# Autodesk Inventor assembly: Lower_Leg_Right
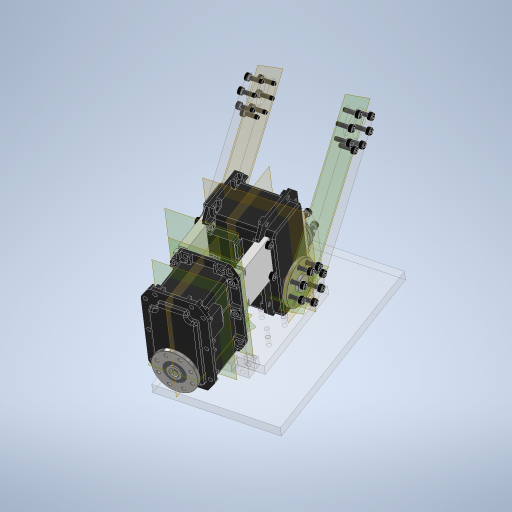
[picture p0: Inventor's stored thumbnail of the model, 512x512]
Saved by Autodesk Inventor 2024 (Build 280153000, 153)
## iProperties
Created: 2024-09-18
Part Number: Lower_Leg_Right
Document SubType Name: Assembly
Designer: Eungang
Author: Eungang
## Documents named in this file (15)
- C:\Users\Eungang\Documents\Inventor\FIGHTING_ROBOT_FINAL\부품\Lower_Leg_Right\Lower_Leg_Right.iam
- C:\Users\Eungang\Documents\Inventor\FIGHTING_ROBOT_FINAL\부품\Lower_Leg_Left\foot_2.ipt
- C:\Users\Eungang\Documents\Inventor\FIGHTING_ROBOT_FINAL\부품\Lower_Leg_Left\foot_ankle_bridge.ipt
- C:\Users\Eungang\Documents\Inventor\FIGHTING_ROBOT_FINAL\부품\Lower_Leg_Left\MX-64T.ipt
- C:\Users\Eungang\Documents\Inventor\FIGHTING_ROBOT_FINAL\부품\혼\64-106Horn.ipt
- C:\Users\Eungang\Documents\Inventor\FIGHTING_ROBOT_FINAL\부품\아이들러\64아이들러.iam
- C:\Users\Eungang\Documents\Inventor\FIGHTING_ROBOT_FINAL\부품\Lower_Leg_Left\MX-106T.ipt
- C:\Users\Eungang\Documents\Inventor\FIGHTING_ROBOT_FINAL\64-106_connect.ipt
- C:\Users\Eungang\Documents\Inventor\FIGHTING_ROBOT_FINAL\부품\Bolt_Washer_Nut\CSH-ST-M2_5-8_203.ipt
- C:\Users\Eungang\Documents\Inventor\FIGHTING_ROBOT_FINAL\부품\Bolt_Washer_Nut\SLBNR2_5.ipt
- C:\Users\Eungang\Documents\Inventor\FIGHTING_ROBOT_FINAL\calf.ipt
- C:\Users\Eungang\Documents\Inventor\FIGHTING_ROBOT_FINAL\부품\Bolt_Washer_Nut\bolt_set_2.5_8 x 7.iam
- C:\Users\Eungang\Documents\Inventor\FIGHTING_ROBOT_FINAL\부품\Lower_Leg_Left\OldVersions\bolt_set_2.5_8 x 7.iam
- C:\Users\Eungang\Documents\Inventor\FIGHTING_ROBOT_FINAL\부품\Lower_Leg_Left\foot_motor_bridge_MIR.ipt
- C:\Users\Eungang\Documents\Inventor\FIGHTING_ROBOT_FINAL\부품\Lower_Leg_Right\foot_1.ipt
## Components (35 placed, 13 different names)
1. foot_2:1 — 삽입:73, 삽입:94, 삽입:95
2. foot_ankle_bridge:2 — 삽입:72, 삽입:82
3. 64-106_connect:1 — 삽입:62, 삽입:63, 삽입:88, 삽입:89
4. bolt_set_2.5_8 x 7:1 [sub-assembly]
5. SLBNR2_5:2
6. CSH-ST-M2_5-8_203:18
7. 64-106_connect:2 — 삽입:60, 삽입:61, 삽입:64, 삽입:65
8. CSH-ST-M2_5-8_203:19
9. CSH-ST-M2_5-8_203:20
10. SLBNR2_5:5
11. SLBNR2_5:6
12. MX-106T:1 — 삽입:54, 삽입:55, 삽입:60, 삽입:61, 삽입:62, 삽입:63, 삽입:69, 삽입:70, 삽입:92, 삽입:93, 메이트:2
13. 64아이들러:2 [sub-assembly] — 삽입:55, 삽입:58, 삽입:59
14. calf:1 — 삽입:56, 삽입:57, 삽입:84, 삽입:85, 각도:2, 삽입:96, 삽입:97
15. bolt_set_2.5_8 x 7:2 [sub-assembly] — 삽입:78, 삽입:79
16. calf:2 — 삽입:58, 삽입:59, 삽입:78, 삽입:79, 삽입:86, 삽입:87, 각도:1
17. 64-106Horn:2 — 삽입:54, 삽입:56, 삽입:57
18. 64-106Horn:3 — 삽입:66, 삽입:68, 삽입:83
19. foot_ankle_bridge:3 — 삽입:68, 삽입:73, 삽입:83
20. MX-64T:1 — 삽입:64, 삽입:65, 삽입:66, 삽입:67, 삽입:80, 삽입:81, 삽입:90, 삽입:91
21. 64아이들러:3 [sub-assembly] — 삽입:67
22. foot_motor_bridge_MIR:1 — 삽입:69, 삽입:70, 삽입:71
23. 64아이들러:4 [sub-assembly] — 삽입:71, 삽입:72, 삽입:82, 메이트:2
24. CSH-ST-M2_5-8_203:21 — 삽입:81
25. CSH-ST-M2_5-8_203:22 — 삽입:80
26. bolt_set_2.5_8 x 7:3 [sub-assembly] — 삽입:86, 삽입:87
27. bolt_set_2.5_8 x 7:4 [sub-assembly] — 삽입:84, 삽입:85
28. CSH-ST-M2_5-8_203:23 — 삽입:88
29. SLBNR2_5:7 — 삽입:89
30. CSH-ST-M2_5-8_203:24 — 삽입:90
31. CSH-ST-M2_5-8_203:25 — 삽입:91
32. SLBNR2_5:8 — 삽입:92
33. SLBNR2_5:9 — 삽입:93
34. foot_1:1 — 삽입:94, 삽입:95, 각도:1, 각도:2
35. bolt_set_2.5_8 x 7:5 [sub-assembly] — 삽입:96, 삽입:97
## Relationships (53: Insert 49, Mate 2, Angle 2)
- [Mate] (0.1 mm): foot_2:1 ↔ foot_ankle_bridge:2
- [Insert]: foot_2:1 ↔ foot_ankle_bridge:2
- [Insert]: foot_ankle_bridge:2 ↔ bolt_set_2.5_8 x 7:1
- [Insert]: foot_ankle_bridge:2 ↔ bolt_set_2.5_8 x 7:1
- [Insert] (0.1 mm): 64-106_connect:1 ↔ SLBNR2_5:2
- [Insert]: 64-106_connect:1 ↔ CSH-ST-M2_5-8_203:18
- [Insert]: 64-106_connect:2 ↔ CSH-ST-M2_5-8_203:20
- [Insert]: 64-106_connect:2 ↔ CSH-ST-M2_5-8_203:19
- [Insert] (0.1 mm): 64-106_connect:2 ↔ SLBNR2_5:5
- [Insert] (0.1 mm): 64-106_connect:2 ↔ SLBNR2_5:6
- 삽입:54 [Insert] (0.5 mm): MX-106T:1 ↔ 64-106Horn:2
- 삽입:55 [Insert] (0.5 mm): MX-106T:1 ↔ 64아이들러:2
- 삽입:56 [Insert]: calf:1 ↔ 64-106Horn:2
- 삽입:57 [Insert]: calf:1 ↔ 64-106Horn:2
- 삽입:58 [Insert]: 64아이들러:2 ↔ calf:2
- 삽입:59 [Insert]: 64아이들러:2 ↔ calf:2
- 삽입:60 [Insert] (0.1 mm): 64-106_connect:2 ↔ MX-106T:1
- 삽입:61 [Insert] (0.1 mm): 64-106_connect:2 ↔ MX-106T:1
- 삽입:62 [Insert] (0.1 mm): 64-106_connect:1 ↔ MX-106T:1
- 삽입:63 [Insert] (0.1 mm): 64-106_connect:1 ↔ MX-106T:1
- 삽입:64 [Insert] (0.1 mm): 64-106_connect:2 ↔ MX-64T:1
- 삽입:65 [Insert] (0.1 mm): 64-106_connect:2 ↔ MX-64T:1
- 삽입:66 [Insert] (0.5 mm): 64-106Horn:3 ↔ MX-64T:1
- 삽입:67 [Insert] (0.5 mm): MX-64T:1 ↔ 64아이들러:3
- 삽입:68 [Insert]: 64-106Horn:3 ↔ foot_ankle_bridge:3
- 삽입:69 [Insert] (0.1 mm): MX-106T:1 ↔ foot_motor_bridge_MIR:1
- 삽입:70 [Insert] (0.1 mm): MX-106T:1 ↔ foot_motor_bridge_MIR:1
- 삽입:71 [Insert]: foot_motor_bridge_MIR:1 ↔ 64아이들러:4
- 삽입:72 [Insert]: foot_ankle_bridge:2 ↔ 64아이들러:4
- 삽입:73 [Insert] (0.1 mm): foot_2:1 ↔ foot_ankle_bridge:3
- 삽입:78 [Insert]: bolt_set_2.5_8 x 7:2 ↔ calf:2
- 삽입:79 [Insert]: bolt_set_2.5_8 x 7:2 ↔ calf:2
- 삽입:80 [Insert]: MX-64T:1 ↔ CSH-ST-M2_5-8_203:22
- 삽입:81 [Insert]: MX-64T:1 ↔ CSH-ST-M2_5-8_203:21
- 삽입:82 [Insert]: foot_ankle_bridge:2 ↔ 64아이들러:4
- 삽입:83 [Insert]: 64-106Horn:3 ↔ foot_ankle_bridge:3
- 삽입:84 [Insert]: calf:1 ↔ bolt_set_2.5_8 x 7:4
- 삽입:85 [Insert]: calf:1 ↔ bolt_set_2.5_8 x 7:4
- 삽입:86 [Insert]: calf:2 ↔ bolt_set_2.5_8 x 7:3
- 삽입:87 [Insert]: calf:2 ↔ bolt_set_2.5_8 x 7:3
- 삽입:88 [Insert]: 64-106_connect:1 ↔ CSH-ST-M2_5-8_203:23
- 삽입:89 [Insert] (0.1 mm): 64-106_connect:1 ↔ SLBNR2_5:7
- 삽입:90 [Insert]: MX-64T:1 ↔ CSH-ST-M2_5-8_203:24
- 삽입:91 [Insert]: MX-64T:1 ↔ CSH-ST-M2_5-8_203:25
- 삽입:92 [Insert]: MX-106T:1 ↔ SLBNR2_5:8
- 삽입:93 [Insert]: MX-106T:1 ↔ SLBNR2_5:9
- 메이트:2 [Mate]: MX-106T:1 ↔ 64아이들러:4
- 삽입:94 [Insert]: foot_2:1 ↔ foot_1:1
- 삽입:95 [Insert]: foot_2:1 ↔ foot_1:1
- 각도:1 [Angle] (135 deg): calf:2 ↔ foot_1:1
- 각도:2 [Angle] (225 deg): calf:1 ↔ foot_1:1
- 삽입:96 [Insert]: calf:1 ↔ bolt_set_2.5_8 x 7:5
- 삽입:97 [Insert]: calf:1 ↔ bolt_set_2.5_8 x 7:5
## Named parameters: d0_d3 = 0.1 mm, d1_d4 = 0 mm
